# Autodesk Inventor assembly: Assembly2
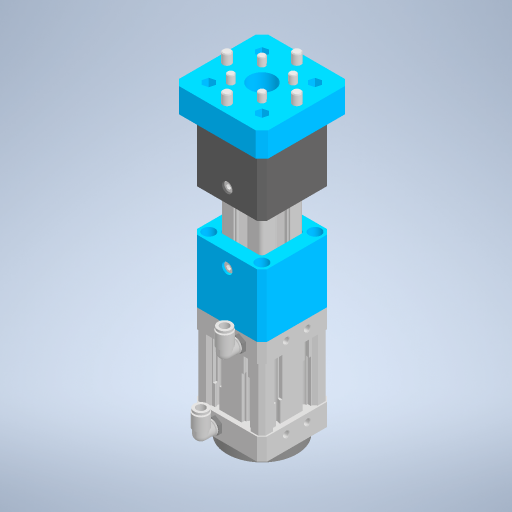
[picture p0: Inventor's stored thumbnail of the model, 512x512]
Saved by Autodesk Inventor 2023 (Build 270158000, 158)
## iProperties
Created: 2022-05-24
Part Number: Assembly2
Document SubType Name: Assembly
Designer: romanp
Author: romanp
## Documents named in this file (13)
- C:\Users\romanp\Desktop\SMC_End_Effector_Prototype\SMC_EE_MHM-32D1-X6400\Pack_and_Go\Assembly_SMC_EE.iam
- C:\Users\romanp\Desktop\SMC_End_Effector_Prototype\SMC_EE_MHM-32D1-X6400\Pack_and_Go\MHM-32D1-X6400(0).iam
- C:\Users\romanp\Desktop\SMC_End_Effector_Prototype\SMC_EE_MHM-32D1-X6400\Pack_and_Go\Part_Top_Blue.ipt
- C:\Users\romanp\Desktop\SMC_End_Effector_Prototype\SMC_EE_MHM-32D1-X6400\Pack_and_Go\Part_Bottom_Blue.ipt
- C:\Users\romanp\Desktop\SMC_End_Effector_Prototype\SMC_EE_MHM-32D1-X6400\Pack_and_Go\Part_Middle_Black.ipt
- C:\Users\romanp\Desktop\SMC_End_Effector_Prototype\SMC_EE_MHM-32D1-X6400\Pack_and_Go\ITEM30x30x100.ipt
- C:\Users\romanp\Desktop\SMC_End_Effector_Prototype\SMC_EE_MHM-32D1-X6400\Pack_and_Go\M4x10.ipt
- C:\Users\romanp\Desktop\SMC_End_Effector_Prototype\SMC_EE_MHM-32D1-X6400\Pack_and_Go\M5x20.ipt
- C:\Users\romanp\Desktop\SMC_End_Effector_Prototype\SMC_EE_MHM-32D1-X6400\Pack_and_Go\KQ2L06-01N.ipt
- C:\Users\romanp\Desktop\SMC_End_Effector_Prototype\SMC_EE_MHM-32D1-X6400\Pack_and_Go\hex_socket_cylindrical_head_M4x25.ipt
- C:\Users\romanp\Desktop\SMC_End_Effector_Prototype\SMC_EE_MHM-32D1-X6400\Pack_and_Go\M4_nut.ipt
- C:\Users\romanp\Desktop\SMC_End_Effector_Prototype\SMC_EE_MHM-32D1-X6400\Pack_and_Go\hex_socket_cylindrical_head_M5x16.ipt
- C:\Users\romanp\Desktop\SMC_End_Effector_Prototype\SMC_EE_MHM-32D1-X6400\Pack_and_Go\hex_socket_cylindrical_head_M6x16.ipt
## Components (31 placed, 12 different names)
1. M4x10:5
2. M4x10:7
3. ITEM30x30x100:3
4. MHM-32D1-X6400(0):3 [sub-assembly] — Insert:51, Insert:52, Insert:53
5. M5x75:2
6. M4x10:8
7. M4x10:9
8. M5x75:3
9. M5x75:4
10. M5x75:5
11. KQ2L06-01N:3 — Insert:51
12. KQ2L06-01N:4 — Insert:52
13. Part_Bottom_Blue:1 — Insert:53
14. Part_Middle_Black:2 — Insert:54, Insert:55, Insert:56, Insert:57, Insert:58
15. Part_Top_Blue:4 — Insert:54, Insert:59, Insert:60, Insert:61, Insert:62, Insert:63, Insert:64, Insert:65, Insert:66, Insert:67, Mate:1, Mate:2, Mate:3
16. M4x25:1 — Insert:55
17. M4x25:2 — Insert:57
18. M4x25:3 — Insert:58
19. M4x25:4 — Insert:56
20. M4_nut:1 — Insert:59
21. M5x16:1 — Insert:63
22. M6x16:1 — Insert:67
23. M4_nut:2 — Insert:62
24. M4_nut:3 — Insert:61
25. M4_nut:4 — Insert:60
26. M5x16:2 — Insert:64
27. M5x16:3 — Insert:65
28. M5x16:4 — Insert:66
29. M6x16:2 — Mate:3
30. M6x16:3 — Mate:2
31. M6x16:4 — Mate:1
## Relationships (20: Insert 17, Mate 3)
- Insert:51: MHM-32D1-X6400(0):3 ↔ KQ2L06-01N:3
- Insert:52: MHM-32D1-X6400(0):3 ↔ KQ2L06-01N:4
- Insert:53: MHM-32D1-X6400(0):3 ↔ Part_Bottom_Blue:1
- Insert:54: Part_Middle_Black:2 ↔ Part_Top_Blue:4
- Insert:55: Part_Middle_Black:2 ↔ M4x25:1
- Insert:56: Part_Middle_Black:2 ↔ M4x25:4
- Insert:57: Part_Middle_Black:2 ↔ M4x25:2
- Insert:58: Part_Middle_Black:2 ↔ M4x25:3
- Insert:59: Part_Top_Blue:4 ↔ M4_nut:1
- Insert:60: Part_Top_Blue:4 ↔ M4_nut:4
- Insert:61: Part_Top_Blue:4 ↔ M4_nut:3
- Insert:62: Part_Top_Blue:4 ↔ M4_nut:2
- Insert:63: Part_Top_Blue:4 ↔ M5x16:1
- Insert:64: Part_Top_Blue:4 ↔ M5x16:2
- Insert:65: Part_Top_Blue:4 ↔ M5x16:3
- Insert:66: Part_Top_Blue:4 ↔ M5x16:4
- Insert:67: Part_Top_Blue:4 ↔ M6x16:1
- Mate:1: Part_Top_Blue:4 ↔ M6x16:4
- Mate:2: Part_Top_Blue:4 ↔ M6x16:3
- Mate:3: Part_Top_Blue:4 ↔ M6x16:2
